# Autodesk Inventor assembly: coxaCircleAssembly
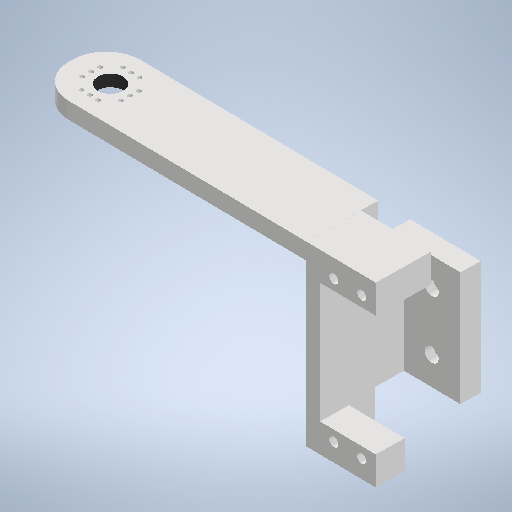
[picture p0: Inventor's stored thumbnail of the model, 512x512]
Saved by Autodesk Inventor 2025.1 (Build 291241020, 241B)
## iProperties
Created: 2024-10-14
Part Number: coxaCircleAssembly
Document SubType Name: Assembly
Designer: omiye
Author: omiye
## Documents named in this file (3)
- C:\Projects\Arduino\hexapod\legModels\miscStuff\coxaCircleAssembly.iam
- C:\Projects\Arduino\hexapod\legModels\coxaModelCircle.ipt
- C:\Projects\Arduino\hexapod\legModels\circleCoxaModel.ipt
## Components (2 placed, 2 different names)
1. coxaModelCircle:1 — Mate:1, Mate:2
2. circleCoxaModel:1 — Mate:1, Mate:2
## Relationships (2: Mate 2)
- Mate:1: coxaModelCircle:1 ↔ circleCoxaModel:1
- Mate:2: coxaModelCircle:1 ↔ circleCoxaModel:1
